# Autodesk Inventor assembly: TL20240901-10320CV-000
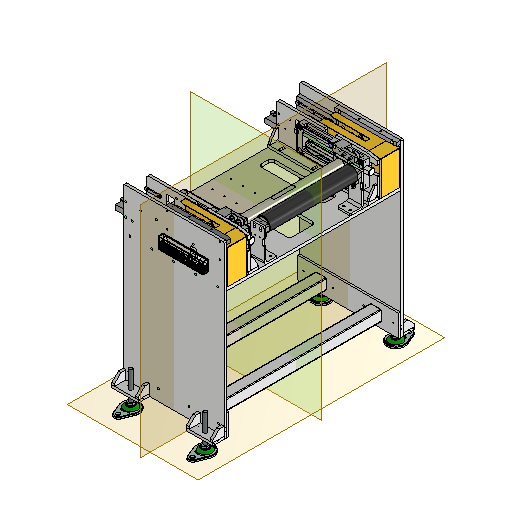
[picture p0: Inventor's stored thumbnail of the model, 512x512]
Saved by Autodesk Inventor 2022.6 (Build 266554000, 554)
## iProperties
Category: CONVEYOR ASSY
Company: 현대 트랜시스
Created: 2023-04-11
Part Number: TL20240901-10320CV-000
Checked By: 김형민
Engr Approved By: 김형민
User Status: 1 x6
Description: 5
Document SubType Name: Assembly
Mfg Approved By: 호상태
Designer: 박성규
Stock Number: 000
Project: MEa-PJT 2LINE
DocNumber: TN20221101-FA000000-000-1.iam
Folder: OLD\개발설비\1. 사내개발\19. 미쓰비시 컨버팅 솔루션 데모장비\
Detail Description: Assembly products
Title: FOLLOWER UNIT ASSY
Subject: MEa차종 시트조립2라인
Author: 박성규
Revision Number: A
## Documents named in this file (45)
- D:\V\Designs\프로젝트 자산\자동화 & 스마트팩토리\현대트랜시스(구 다이모스, 파워텍)\트랜시스(사바나)_TL20240901-MEa차종 시트조립2라인 조립컨베어 신작\2. 제작도면\1열\10300CV(CONVEYOR)\10320CV(FOLLOWER UNIT)\TL20240901-10320CV-000.iam
- D:\V\Designs\프로젝트 자산\자동화 & 스마트팩토리\현대트랜시스(구 다이모스, 파워텍)\트랜시스(사바나)_TL20240901-MEa차종 시트조립2라인 조립컨베어 신작\2. 제작도면\1열\10300CV(CONVEYOR)\10320CV(FOLLOWER UNIT)\TL20240901-10320CV-005.ipt
- D:\V\Designs\프로젝트 자산\자동화 & 스마트팩토리\현대트랜시스(구 다이모스, 파워텍)\트랜시스(사바나)_TL20240901-MEa차종 시트조립2라인 조립컨베어 신작\2. 제작도면\1열\10300CV(CONVEYOR)\10320CV(FOLLOWER UNIT)\TL20240901-10320CV-019.ipt
- D:\V\Designs\프로젝트 자산\자동화 & 스마트팩토리\현대트랜시스(구 다이모스, 파워텍)\트랜시스(사바나)_TL20240901-MEa차종 시트조립2라인 조립컨베어 신작\2. 제작도면\1열\10300CV(CONVEYOR)\10320CV(FOLLOWER UNIT)\TL20240901-10320CV-015.ipt
- D:\V\Designs\프로젝트 자산\자동화 & 스마트팩토리\현대트랜시스(구 다이모스, 파워텍)\트랜시스(사바나)_TL20240901-MEa차종 시트조립2라인 조립컨베어 신작\2. 제작도면\1열\10300CV(CONVEYOR)\10320CV(FOLLOWER UNIT)\TL20240901-10320CV-001.ipt
- D:\V\Designs\프로젝트 자산\자동화 & 스마트팩토리\현대트랜시스(구 다이모스, 파워텍)\트랜시스(사바나)_TL20240901-MEa차종 시트조립2라인 조립컨베어 신작\2. 제작도면\1열\10300CV(CONVEYOR)\10320CV(FOLLOWER UNIT)\TL20240901-10320CV-002.ipt
- D:\V\Designs\프로젝트 자산\자동화 & 스마트팩토리\현대트랜시스(구 다이모스, 파워텍)\트랜시스(사바나)_TL20240901-MEa차종 시트조립2라인 조립컨베어 신작\2. 제작도면\1열\10300CV(CONVEYOR)\10320CV(FOLLOWER UNIT)\TL20240901-10320CV-024.ipt
- D:\V\Designs\프로젝트 자산\자동화 & 스마트팩토리\현대트랜시스(구 다이모스, 파워텍)\트랜시스(사바나)_TL20240901-MEa차종 시트조립2라인 조립컨베어 신작\2. 제작도면\1열\10300CV(CONVEYOR)\10320CV(FOLLOWER UNIT)\TL20240901-10320CV-013.ipt
- D:\V\Designs\구매품(업체별)\THK\CAM FOLLOWER_CF10-1UU_THK.ipt
- D:\V\Designs\구매품(업체별)\BUYOUNG\ADJUST ANCHOR_BYARB-81-M16X130_BUYOUNG.ipt
- D:\V\Designs\프로젝트 자산\자동화 & 스마트팩토리\현대트랜시스(구 다이모스, 파워텍)\트랜시스(사바나)_TL20240901-MEa차종 시트조립2라인 조립컨베어 신작\2. 제작도면\1열\10300CV(CONVEYOR)\10320CV(FOLLOWER UNIT)\TL20240901-10320CV-014.ipt
- D:\V\Designs\프로젝트 자산\자동화 & 스마트팩토리\현대트랜시스(구 다이모스, 파워텍)\트랜시스(사바나)_TL20240901-MEa차종 시트조립2라인 조립컨베어 신작\2. 제작도면\1열\10300CV(CONVEYOR)\10320CV(FOLLOWER UNIT)\TL20240901-10320CV-014-MIR.ipt
- D:\V\Designs\프로젝트 자산\자동화 & 스마트팩토리\현대트랜시스(구 다이모스, 파워텍)\트랜시스(사바나)_TL20240901-MEa차종 시트조립2라인 조립컨베어 신작\2. 제작도면\1열\10300CV(CONVEYOR)\10320CV(FOLLOWER UNIT)\TL20240901-10320CV-022.ipt
- D:\V\Designs\프로젝트 자산\자동화 & 스마트팩토리\현대트랜시스(구 다이모스, 파워텍)\트랜시스(사바나)_TL20240901-MEa차종 시트조립2라인 조립컨베어 신작\2. 제작도면\1열\10300CV(CONVEYOR)\10320CV(FOLLOWER UNIT)\TL20240901-10320CV-023.ipt
- D:\V\Designs\구매품(업체별)\EUNHYUN\FREE ROLLER_FR570-400-12-JD-ZN-NR630A_EUNHYUN.ipt
- D:\V\Designs\프로젝트 자산\자동화 & 스마트팩토리\현대트랜시스(구 다이모스, 파워텍)\트랜시스(사바나)_TL20240901-MEa차종 시트조립2라인 조립컨베어 신작\2. 제작도면\1열\10300CV(CONVEYOR)\10320CV(FOLLOWER UNIT)\TL20240901-10320CV-008.ipt
- D:\V\Designs\프로젝트 자산\자동화 & 스마트팩토리\현대트랜시스(구 다이모스, 파워텍)\트랜시스(사바나)_TL20240901-MEa차종 시트조립2라인 조립컨베어 신작\2. 제작도면\1열\10300CV(CONVEYOR)\10320CV(FOLLOWER UNIT)\TL20240901-10320CV-007.ipt
- D:\V\Designs\구매품(업체별)\NSK\BEARING_60-32ZZ_NSK.ipt
- D:\V\Designs\프로젝트 자산\자동화 & 스마트팩토리\현대트랜시스(구 다이모스, 파워텍)\트랜시스(사바나)_TL20240901-MEa차종 시트조립2라인 조립컨베어 신작\2. 제작도면\1열\10300CV(CONVEYOR)\10320CV(FOLLOWER UNIT)\TL20240901-10320CV-010.ipt
- D:\V\Designs\프로젝트 자산\자동화 & 스마트팩토리\현대트랜시스(구 다이모스, 파워텍)\트랜시스(사바나)_TL20240901-MEa차종 시트조립2라인 조립컨베어 신작\2. 제작도면\1열\10300CV(CONVEYOR)\10320CV(FOLLOWER UNIT)\TL20240901-10320CV-006.ipt
- D:\V\Designs\프로젝트 자산\자동화 & 스마트팩토리\현대트랜시스(구 다이모스, 파워텍)\트랜시스(사바나)_TL20240901-MEa차종 시트조립2라인 조립컨베어 신작\2. 제작도면\1열\10300CV(CONVEYOR)\10320CV(FOLLOWER UNIT)\TL20240901-10320CV-009.ipt
- D:\V\Designs\프로젝트 자산\자동화 & 스마트팩토리\현대트랜시스(구 다이모스, 파워텍)\트랜시스(사바나)_TL20240901-MEa차종 시트조립2라인 조립컨베어 신작\2. 제작도면\1열\10300CV(CONVEYOR)\10320CV(FOLLOWER UNIT)\TL20240901-10320CV-002-MIR.ipt
- D:\V\Designs\프로젝트 자산\자동화 & 스마트팩토리\현대트랜시스(구 다이모스, 파워텍)\트랜시스(사바나)_TL20240901-MEa차종 시트조립2라인 조립컨베어 신작\2. 제작도면\1열\10300CV(CONVEYOR)\10320CV(FOLLOWER UNIT)\TL20240901-10320CV-005-MIR.ipt
- D:\V\Designs\프로젝트 자산\자동화 & 스마트팩토리\현대트랜시스(구 다이모스, 파워텍)\트랜시스(사바나)_TL20240901-MEa차종 시트조립2라인 조립컨베어 신작\2. 제작도면\1열\10300CV(CONVEYOR)\10320CV(FOLLOWER UNIT)\TL20240901-10320CV-011.ipt
- D:\V\Designs\구매품(업체별)\기타\TAKE UP UNIT_CTSN-9(L)_SHINWOO.iam
- D:\V\Designs\구매품(업체별)\기타\TAKE UP UNIT_CTSN-9_SHINWOO.iam
- D:\V\Designs\프로젝트 자산\자동화 & 스마트팩토리\현대트랜시스(구 다이모스, 파워텍)\트랜시스(사바나)_TL20240901-MEa차종 시트조립2라인 조립컨베어 신작\2. 제작도면\1열\10300CV(CONVEYOR)\10320CV(FOLLOWER UNIT)\TL20240901-10320CV-012.ipt
- D:\V\Content Center Files\en-US\AS 1420\AS 1420 - 1973 - M8 x 40.ipt
- D:\V\Designs\구매품(업체별)\MISUMI\ADJUST BLOCK_SNTBM8-8_MISUMI.ipt
- D:\V\Content Center Files\en-US\ANSI B 18.2.4.1 M(1)\ANSI B 18.2.4.1 M - M8 x 1.25Style 1.ipt
- D:\V\Designs\프로젝트 자산\자동화 & 스마트팩토리\현대트랜시스(구 다이모스, 파워텍)\트랜시스(사바나)_TL20240901-MEa차종 시트조립2라인 조립컨베어 신작\2. 제작도면\1열\10300CV(CONVEYOR)\10320CV(FOLLOWER UNIT)\TL20240901-10320CV-020.ipt
- D:\V\Designs\프로젝트 자산\자동화 & 스마트팩토리\현대트랜시스(구 다이모스, 파워텍)\트랜시스(사바나)_TL20240901-MEa차종 시트조립2라인 조립컨베어 신작\2. 제작도면\1열\10300CV(CONVEYOR)\10320CV(FOLLOWER UNIT)\TL20240901-10320CV-016.ipt
- D:\V\Designs\프로젝트 자산\자동화 & 스마트팩토리\현대트랜시스(구 다이모스, 파워텍)\트랜시스(사바나)_TL20240901-MEa차종 시트조립2라인 조립컨베어 신작\2. 제작도면\1열\10300CV(CONVEYOR)\10320CV(FOLLOWER UNIT)\TL20240901-10320CV-016-MIR.ipt
- D:\V\Designs\프로젝트 자산\자동화 & 스마트팩토리\현대트랜시스(구 다이모스, 파워텍)\트랜시스(사바나)_TL20240901-MEa차종 시트조립2라인 조립컨베어 신작\2. 제작도면\1열\10300CV(CONVEYOR)\10320CV(FOLLOWER UNIT)\TL20240901-10320CV-017.ipt
- D:\V\Designs\프로젝트 자산\자동화 & 스마트팩토리\현대트랜시스(구 다이모스, 파워텍)\트랜시스(사바나)_TL20240901-MEa차종 시트조립2라인 조립컨베어 신작\2. 제작도면\1열\10300CV(CONVEYOR)\10320CV(FOLLOWER UNIT)\TL20240901-10320CV-018.ipt
- D:\V\Designs\프로젝트 자산\자동화 & 스마트팩토리\현대트랜시스(구 다이모스, 파워텍)\트랜시스(사바나)_TL20240901-MEa차종 시트조립2라인 조립컨베어 신작\2. 제작도면\1열\10300CV(CONVEYOR)\10320CV(FOLLOWER UNIT)\TL20240901-10320CV-004.ipt
- D:\V\Designs\프로젝트 자산\자동화 & 스마트팩토리\현대트랜시스(구 다이모스, 파워텍)\트랜시스(사바나)_TL20240901-MEa차종 시트조립2라인 조립컨베어 신작\2. 제작도면\1열\10300CV(CONVEYOR)\10320CV(FOLLOWER UNIT)\TL20240901-10320CV-003.ipt
- D:\V\Designs\프로젝트 자산\자동화 & 스마트팩토리\현대트랜시스(구 다이모스, 파워텍)\트랜시스(사바나)_TL20240901-MEa차종 시트조립2라인 조립컨베어 신작\2. 제작도면\1열\10300CV(CONVEYOR)\10320CV(FOLLOWER UNIT)\TL20240901-10320CV-013-MIR.ipt
- D:\V\Designs\프로젝트 자산\자동화 & 스마트팩토리\현대트랜시스(구 다이모스, 파워텍)\트랜시스(사바나)_TL20240901-MEa차종 시트조립2라인 조립컨베어 신작\2. 제작도면\1열\10300CV(CONVEYOR)\10320CV(FOLLOWER UNIT)\TL20240901-10320CV-021.ipt
- D:\V\Designs\구매품(업체별)\OMRON\PROXIMITY SENSOR_E2B-M18KS08-WP-B1_OMRON.ipt
- D:\V\Designs\구매품(업체별)\BUYOUNG\END CAP_BYEC-2020P-BK_BUYOUNG.ipt
- D:\V\Designs\프로젝트 자산\자동화 & 스마트팩토리\현대트랜시스(구 다이모스, 파워텍)\트랜시스(사바나)_TL20240901-MEa차종 시트조립2라인 조립컨베어 신작\2. 제작도면\1열\10300CV(CONVEYOR)\10320CV(FOLLOWER UNIT)\TL20240901-10320CV-025.ipt
- D:\V\Designs\프로젝트 자산\자동화 & 스마트팩토리\현대트랜시스(구 다이모스, 파워텍)\트랜시스(사바나)_TL20240901-MEa차종 시트조립2라인 조립컨베어 신작\2. 제작도면\1열\10300CV(CONVEYOR)\10320CV(FOLLOWER UNIT)\TL20240901-10320CV-027.ipt
- D:\V\Designs\프로젝트 자산\자동화 & 스마트팩토리\현대트랜시스(구 다이모스, 파워텍)\트랜시스(사바나)_TL20240901-MEa차종 시트조립2라인 조립컨베어 신작\2. 제작도면\1열\10300CV(CONVEYOR)\10320CV(FOLLOWER UNIT)\TL20240901-10320CV-026.ipt
- D:\V\Designs\프로젝트 자산\자동화 & 스마트팩토리\현대트랜시스(구 다이모스, 파워텍)\트랜시스(사바나)_TL20240901-MEa차종 시트조립2라인 조립컨베어 신작\2. 제작도면\1열\10300CV(CONVEYOR)\10320CV(FOLLOWER UNIT)\TL20240901-10320CV-101.ipt
## Components (96 placed, 44 different names)
1. ADJUST ANCHOR_BYARB-81-M16X130_BUYOUNG.ipt:1 — 메이트:426, 플러쉬:20, 플러쉬:21, 각도:2, 각도:3, Flush:44
2. ADJUST ANCHOR_BYARB-81-M16X130_BUYOUNG.ipt:2 — 메이트:427, 플러쉬:21, 각도:3
3. ADJUST ANCHOR_BYARB-81-M16X130_BUYOUNG.ipt:3 — 메이트:424, 플러쉬:19, 플러쉬:20, 각도:5, Flush:22, Flush:44
4. ADJUST ANCHOR_BYARB-81-M16X130_BUYOUNG.ipt:4 — 메이트:425, 플러쉬:19, 각도:5, Mate:518
5. ADJUST BLOCK_SNTBM8-8_MISUMI.ipt:1 — Mate:586, Mate:587, Mate:588, Mate:589, Mate:590
6. ADJUST BLOCK_SNTBM8-8_MISUMI.ipt:2 — Mate:594, Mate:595, Mate:596
7. ANSI B 18.2.4.1 M - M8 x 1.25Style 1.ipt:1 — Mate:590
8. ANSI B 18.2.4.1 M - M8 x 1.25Style 1.ipt:2
9. AS 1420 - 1973 - M8 x 40.ipt:1 — Mate:589
10. AS 1420 - 1973 - M8 x 40.ipt:2 — Mate:597
11. BEARING_60-32ZZ_NSK.ipt:1
12. BEARING_60-32ZZ_NSK.ipt:2
13. BEARING_60-32ZZ_NSK.ipt:3
14. BEARING_60-32ZZ_NSK.ipt:4
15. CAM FOLLOWER_CF10-1UU_THK.ipt:1
16. CAM FOLLOWER_CF10-1UU_THK.ipt:2
17. CAM FOLLOWER_CF10-1UU_THK.ipt:3 — Mate:599, Mate:604
18. CAM FOLLOWER_CF10-1UU_THK.ipt:4 — Mate:598, Mate:603
19. END CAP_BYEC-2020P-BK_BUYOUNG.ipt:1
20. END CAP_BYEC-2020P-BK_BUYOUNG.ipt:2
21. END CAP_BYEC-2020P-BK_BUYOUNG.ipt:3
22. END CAP_BYEC-2020P-BK_BUYOUNG.ipt:4
23. FREE ROLLER_FR570-400-12-JD-ZN-NR630A_EUNHYUN.ipt:1
24. PROXIMITY SENSOR_E2B-M18KS08-WP-B1_OMRON.ipt:1
25. PROXIMITY SENSOR_E2B-M18KS08-WP-B1_OMRON.ipt:2
26. TAKE UP UNIT_CTSN-9(L)_SHINWOO.iam:1 [sub-assembly] — Mate:561, Mate:562, Mate:563, Mate:564, Mate:566, Mate:567, Mate:568, Mate:569, Mate:574, Mate:585
27. TAKE UP UNIT_CTSN-9_SHINWOO.iam:1 [sub-assembly] — Mate:565, Mate:570, Mate:571, Mate:572, Mate:573, Mate:584
28. TL20240901-10320CV-001.ipt:1 — 메이트:148, 메이트:149, 메이트:150, 메이트:194, Mate:451, Mate:452, Mate:473, Mate:508, Mate:509, Mate:510, Mate:529, Mate:530, Mate:531, Mate:532, Mate:575, Mate:580, Flush:41, Mate:582, Flush:42, Angle:6, Angle:7
29. TL20240901-10320CV-002-MIR.ipt:1 — Mate:499, Mate:500, Mate:501, Mate:502, Mate:503, Mate:504, Mate:505, Mate:506, Mate:507, Mate:508, Mate:509, Mate:510, Mate:511, Mate:512, Mate:513, Mate:514, Mate:515, Mate:516, Mate:517, Mate:519, Mate:520, Mate:581, Mate:635, Mate:636, Mate:637
30. TL20240901-10320CV-002.ipt:1 — 메이트:148, 메이트:149, 메이트:150, 메이트:206, 메이트:207, 메이트:208, 메이트:209, 메이트:210, 메이트:211, 메이트:378, 메이트:379, 메이트:380, 메이트:389, 메이트:390, 메이트:391, 각도:2, Mate:446, Mate:447, Mate:448, Mate:583, Mate:622, Mate:623, Mate:624
31. TL20240901-10320CV-003.ipt:1
32. TL20240901-10320CV-003.ipt:2
33. TL20240901-10320CV-003.ipt:3
34. TL20240901-10320CV-003.ipt:4 — 메이트:389
35. TL20240901-10320CV-003.ipt:5
36. TL20240901-10320CV-003.ipt:6 — Mate:499
37. TL20240901-10320CV-003.ipt:7
38. TL20240901-10320CV-003.ipt:8
39. TL20240901-10320CV-004.ipt:1 — 메이트:378, 메이트:379, 메이트:380, 메이트:426
40. TL20240901-10320CV-004.ipt:2 — 메이트:390, 메이트:391, 메이트:427
41. TL20240901-10320CV-004.ipt:3 — 메이트:424, Flush:22, Mate:506, Mate:507
42. TL20240901-10320CV-004.ipt:4 — 메이트:425, Mate:503, Mate:504, Mate:505
43. TL20240901-10320CV-005-MIR.ipt:1 — Mate:529, Mate:530, Mate:531, Mate:532, Mate:533, Mate:534, Mate:535, Mate:536, Mate:537, Mate:566, Mate:567, Mate:568, Mate:600, Mate:601, Mate:602
44. TL20240901-10320CV-005.ipt:1 — 메이트:194, 메이트:366, 메이트:367, Mate:451, Mate:452, Mate:528, Mate:565, Mate:570, Mate:571, Mate:605
45. TL20240901-10320CV-006.ipt:1
46. TL20240901-10320CV-006.ipt:2
47. TL20240901-10320CV-007.ipt:1 — Flush:43, Angle:7
48. TL20240901-10320CV-007.ipt:2 — Flush:43
49. TL20240901-10320CV-008.ipt:1 — Mate:572, Mate:574, Mate:575, Mate:584, Angle:6
50. TL20240901-10320CV-009.ipt:1
51. TL20240901-10320CV-009.ipt:2
52. TL20240901-10320CV-010.ipt:1 — Mate:585
53. TL20240901-10320CV-010.ipt:2 — Mate:573
54. TL20240901-10320CV-011.ipt:1
55. TL20240901-10320CV-011.ipt:2 — Mate:563, Mate:564
56. TL20240901-10320CV-011.ipt:3
57. TL20240901-10320CV-011.ipt:4
58. TL20240901-10320CV-011.ipt:5
59. TL20240901-10320CV-011.ipt:6 — Mate:569
60. TL20240901-10320CV-011.ipt:7
61. TL20240901-10320CV-011.ipt:8 — Mate:561, Mate:562
62. TL20240901-10320CV-012.ipt:1
63. TL20240901-10320CV-012.ipt:2
64. TL20240901-10320CV-013-MIR.ipt:1 — Mate:598, Mate:599, Mate:600, Mate:601, Mate:602, Mate:603, Mate:604
65. TL20240901-10320CV-013.ipt:1 — 메이트:366, 메이트:367, Mate:528
66. TL20240901-10320CV-014-MIR.ipt:1 — Mate:446, Mate:447, Mate:448
67. TL20240901-10320CV-014.ipt:1 — Mate:511, Mate:512, Mate:513
68. TL20240901-10320CV-015.ipt:1 — Mate:514, Mate:515, Mate:516
69. TL20240901-10320CV-015.ipt:2 — 메이트:209, 메이트:210, 메이트:211
70. TL20240901-10320CV-016-MIR.ipt:1 — 메이트:206, 메이트:207, 메이트:208
71. TL20240901-10320CV-016.ipt:1 — Mate:517, Mate:519, Mate:520
72. TL20240901-10320CV-017.ipt:1
73. TL20240901-10320CV-017.ipt:2
74. TL20240901-10320CV-018.ipt:1
75. TL20240901-10320CV-018.ipt:2 — Mate:536, Mate:537
76. TL20240901-10320CV-018.ipt:3
77. TL20240901-10320CV-018.ipt:4
78. TL20240901-10320CV-019.ipt:1 — Mate:605
79. TL20240901-10320CV-019.ipt:2 — Mate:533, Mate:534, Mate:535
80. TL20240901-10320CV-020.ipt:1
81. TL20240901-10320CV-020.ipt:2
82. TL20240901-10320CV-021.ipt:1 — Mate:580, Mate:581, Flush:41, Mate:607, Mate:608, Mate:609
83. TL20240901-10320CV-021.ipt:2 — Mate:582, Mate:583, Flush:42, Mate:606, Mate:610, Mate:611
84. TL20240901-10320CV-022.ipt:1 — Mate:473, Mate:586, Mate:587, Mate:588
85. TL20240901-10320CV-022.ipt:2 — Mate:594, Mate:595, Mate:596
86. TL20240901-10320CV-023.ipt:1
87. TL20240901-10320CV-023.ipt:2 — Mate:597
88. TL20240901-10320CV-024.ipt:1 — Flush:39, Flush:40, Mate:500, Mate:501, Mate:502
89. TL20240901-10320CV-025.ipt:1 — Mate:607, Mate:608, Mate:609
90. TL20240901-10320CV-025.ipt:2 — Mate:606, Mate:610, Mate:611
91. TL20240901-10320CV-026.ipt:1 — Flush:51
92. TL20240901-10320CV-026.ipt:2 — Flush:51
93. TL20240901-10320CV-027.ipt:1
94. TL20240901-10320CV-027.ipt:2
95. TL20240901-10320CV-101.ipt:1 — Mate:622, Mate:623, Mate:624
96. TL20240901-10320CV-101.ipt:2 — Mate:635, Mate:636, Mate:637
## Relationships (260: Mate 229, Flush 24, Angle 7)
- 메이트:148 [Mate]: TL20240901-10320CV-001.ipt:1 ↔ TL20240901-10320CV-002.ipt:1
- 메이트:149 [Mate]: TL20240901-10320CV-001.ipt:1 ↔ TL20240901-10320CV-002.ipt:1
- 메이트:150 [Mate]: TL20240901-10320CV-001.ipt:1 ↔ TL20240901-10320CV-002.ipt:1
- [Mate] (5 mm): TL20240901-10320CV-016.ipt:1 ↔ TL20240901-10320CV-018.ipt:4
- [Mate]: TL20240901-10320CV-016.ipt:1 ↔ TL20240901-10320CV-018.ipt:4
- [Mate]: TL20240901-10320CV-016.ipt:1 ↔ TL20240901-10320CV-018.ipt:4
- [Mate] (5 mm): TL20240901-10320CV-016.ipt:1 ↔ TL20240901-10320CV-017.ipt:1
- [Mate]: TL20240901-10320CV-016.ipt:1 ↔ TL20240901-10320CV-017.ipt:1
- [Mate]: TL20240901-10320CV-016.ipt:1 ↔ TL20240901-10320CV-017.ipt:1
- [Mate] (5 mm): TL20240901-10320CV-005.ipt:1 ↔ TL20240901-10320CV-019.ipt:1
- [Mate]: TL20240901-10320CV-005.ipt:1 ↔ TL20240901-10320CV-019.ipt:1
- [Mate] (5 mm): TL20240901-10320CV-005.ipt:1 ↔ TL20240901-10320CV-018.ipt:1
- [Mate]: TL20240901-10320CV-005.ipt:1 ↔ TL20240901-10320CV-018.ipt:1
- [Mate]: TL20240901-10320CV-005.ipt:1 ↔ TL20240901-10320CV-018.ipt:1
- [Mate] (5 mm): TL20240901-10320CV-016-MIR.ipt:1 ↔ TL20240901-10320CV-018.ipt:3
- [Mate] (5 mm): TL20240901-10320CV-016-MIR.ipt:1 ↔ TL20240901-10320CV-017.ipt:2
- [Mate]: TL20240901-10320CV-016-MIR.ipt:1 ↔ TL20240901-10320CV-018.ipt:3
- [Mate]: TL20240901-10320CV-016-MIR.ipt:1 ↔ TL20240901-10320CV-018.ipt:3
- [Mate]: TL20240901-10320CV-016-MIR.ipt:1 ↔ TL20240901-10320CV-017.ipt:2
- [Mate]: TL20240901-10320CV-016-MIR.ipt:1 ↔ TL20240901-10320CV-017.ipt:2
- 메이트:194 [Mate]: TL20240901-10320CV-001.ipt:1 ↔ TL20240901-10320CV-005.ipt:1
- [Mate]: TL20240901-10320CV-001.ipt:1 ↔ TL20240901-10320CV-022.ipt:1
- [Mate]: TL20240901-10320CV-001.ipt:1 ↔ TL20240901-10320CV-022.ipt:2
- 메이트:206 [Mate]: TL20240901-10320CV-002.ipt:1 ↔ TL20240901-10320CV-016-MIR.ipt:1
- 메이트:207 [Mate]: TL20240901-10320CV-002.ipt:1 ↔ TL20240901-10320CV-016-MIR.ipt:1
- 메이트:208 [Mate]: TL20240901-10320CV-002.ipt:1 ↔ TL20240901-10320CV-016-MIR.ipt:1
- 메이트:209 [Mate]: TL20240901-10320CV-002.ipt:1 ↔ TL20240901-10320CV-015.ipt:2
- 메이트:210 [Mate]: TL20240901-10320CV-002.ipt:1 ↔ TL20240901-10320CV-015.ipt:2
- 메이트:211 [Mate]: TL20240901-10320CV-002.ipt:1 ↔ TL20240901-10320CV-015.ipt:2
- [Mate]: CAM FOLLOWER_CF10-1UU_THK.ipt:1 ↔ TL20240901-10320CV-013.ipt:1
- [Mate]: CAM FOLLOWER_CF10-1UU_THK.ipt:1 ↔ TL20240901-10320CV-013.ipt:1
- [Mate]: CAM FOLLOWER_CF10-1UU_THK.ipt:2 ↔ TL20240901-10320CV-013.ipt:1
- [Mate]: CAM FOLLOWER_CF10-1UU_THK.ipt:2 ↔ TL20240901-10320CV-013.ipt:1
- 메이트:366 [Mate]: TL20240901-10320CV-005.ipt:1 ↔ TL20240901-10320CV-013.ipt:1
- 메이트:367 [Mate]: TL20240901-10320CV-005.ipt:1 ↔ TL20240901-10320CV-013.ipt:1
- [Mate]: TL20240901-10320CV-003.ipt:1 ↔ TL20240901-10320CV-004.ipt:1
- [Mate]: TL20240901-10320CV-003.ipt:1 ↔ TL20240901-10320CV-004.ipt:1
- [Mate]: TL20240901-10320CV-003.ipt:1 ↔ TL20240901-10320CV-004.ipt:1
- [Mate]: TL20240901-10320CV-003.ipt:2 ↔ TL20240901-10320CV-004.ipt:1
- [Mate]: TL20240901-10320CV-003.ipt:2 ↔ TL20240901-10320CV-004.ipt:1
- [Mate]: TL20240901-10320CV-003.ipt:2 ↔ TL20240901-10320CV-004.ipt:1
- 메이트:378 [Mate]: TL20240901-10320CV-002.ipt:1 ↔ TL20240901-10320CV-004.ipt:1
- 메이트:379 [Mate]: TL20240901-10320CV-002.ipt:1 ↔ TL20240901-10320CV-004.ipt:1
- 메이트:380 [Mate]: TL20240901-10320CV-002.ipt:1 ↔ TL20240901-10320CV-004.ipt:1
- [Mate]: TL20240901-10320CV-003.ipt:3 ↔ TL20240901-10320CV-004.ipt:2
- [Mate]: TL20240901-10320CV-003.ipt:3 ↔ TL20240901-10320CV-004.ipt:2
- [Mate]: TL20240901-10320CV-003.ipt:3 ↔ TL20240901-10320CV-004.ipt:2
- [Mate]: TL20240901-10320CV-003.ipt:4 ↔ TL20240901-10320CV-004.ipt:2
- [Mate]: TL20240901-10320CV-003.ipt:4 ↔ TL20240901-10320CV-004.ipt:2
- [Mate]: TL20240901-10320CV-003.ipt:4 ↔ TL20240901-10320CV-004.ipt:2
- 메이트:389 [Mate]: TL20240901-10320CV-002.ipt:1 ↔ TL20240901-10320CV-003.ipt:4
- 메이트:390 [Mate]: TL20240901-10320CV-002.ipt:1 ↔ TL20240901-10320CV-004.ipt:2
- 메이트:391 [Mate]: TL20240901-10320CV-002.ipt:1 ↔ TL20240901-10320CV-004.ipt:2
- [Mate]: TL20240901-10320CV-003.ipt:5 ↔ TL20240901-10320CV-004.ipt:3
- [Mate]: TL20240901-10320CV-003.ipt:5 ↔ TL20240901-10320CV-004.ipt:3
- [Mate]: TL20240901-10320CV-003.ipt:5 ↔ TL20240901-10320CV-004.ipt:3
- [Mate]: TL20240901-10320CV-003.ipt:6 ↔ TL20240901-10320CV-004.ipt:3
- [Mate]: TL20240901-10320CV-003.ipt:6 ↔ TL20240901-10320CV-004.ipt:3
- [Mate]: TL20240901-10320CV-003.ipt:6 ↔ TL20240901-10320CV-004.ipt:3
- [Mate]: TL20240901-10320CV-003.ipt:7 ↔ TL20240901-10320CV-004.ipt:4
- [Mate]: TL20240901-10320CV-003.ipt:7 ↔ TL20240901-10320CV-004.ipt:4
- [Mate]: TL20240901-10320CV-003.ipt:7 ↔ TL20240901-10320CV-004.ipt:4
- [Mate]: TL20240901-10320CV-003.ipt:8 ↔ TL20240901-10320CV-004.ipt:4
- [Mate]: TL20240901-10320CV-003.ipt:8 ↔ TL20240901-10320CV-004.ipt:4
- [Mate]: TL20240901-10320CV-003.ipt:8 ↔ TL20240901-10320CV-004.ipt:4
- 메이트:424 [Mate]: ADJUST ANCHOR_BYARB-81-M16X130_BUYOUNG.ipt:3 ↔ TL20240901-10320CV-004.ipt:3
- 메이트:425 [Mate]: ADJUST ANCHOR_BYARB-81-M16X130_BUYOUNG.ipt:4 ↔ TL20240901-10320CV-004.ipt:4
- 플러쉬:19 [Flush]: ADJUST ANCHOR_BYARB-81-M16X130_BUYOUNG.ipt:3 ↔ ADJUST ANCHOR_BYARB-81-M16X130_BUYOUNG.ipt:4
- 메이트:426 [Mate]: ADJUST ANCHOR_BYARB-81-M16X130_BUYOUNG.ipt:1 ↔ TL20240901-10320CV-004.ipt:1
- 플러쉬:20 [Flush]: ADJUST ANCHOR_BYARB-81-M16X130_BUYOUNG.ipt:1 ↔ ADJUST ANCHOR_BYARB-81-M16X130_BUYOUNG.ipt:3
- 메이트:427 [Mate]: ADJUST ANCHOR_BYARB-81-M16X130_BUYOUNG.ipt:2 ↔ TL20240901-10320CV-004.ipt:2
- 플러쉬:21 [Flush]: ADJUST ANCHOR_BYARB-81-M16X130_BUYOUNG.ipt:1 ↔ ADJUST ANCHOR_BYARB-81-M16X130_BUYOUNG.ipt:2
- 각도:2 [Angle] (180 deg): ADJUST ANCHOR_BYARB-81-M16X130_BUYOUNG.ipt:1 ↔ TL20240901-10320CV-002.ipt:1
- 각도:3 [Angle] (0 deg): ADJUST ANCHOR_BYARB-81-M16X130_BUYOUNG.ipt:1 ↔ ADJUST ANCHOR_BYARB-81-M16X130_BUYOUNG.ipt:2
- 각도:5 [Angle] (0 deg): ADJUST ANCHOR_BYARB-81-M16X130_BUYOUNG.ipt:3 ↔ ADJUST ANCHOR_BYARB-81-M16X130_BUYOUNG.ipt:4
- Flush:22 (66 mm): ADJUST ANCHOR_BYARB-81-M16X130_BUYOUNG.ipt:3 ↔ TL20240901-10320CV-004.ipt:3
- Mate:446: TL20240901-10320CV-002.ipt:1 ↔ TL20240901-10320CV-014-MIR.ipt:1
- Mate:447: TL20240901-10320CV-002.ipt:1 ↔ TL20240901-10320CV-014-MIR.ipt:1
- Mate:448: TL20240901-10320CV-002.ipt:1 ↔ TL20240901-10320CV-014-MIR.ipt:1
- Mate:451: TL20240901-10320CV-001.ipt:1 ↔ TL20240901-10320CV-005.ipt:1
- Mate:452: TL20240901-10320CV-001.ipt:1 ↔ TL20240901-10320CV-005.ipt:1
- [Mate]: TL20240901-10320CV-022.ipt:1 ↔ TL20240901-10320CV-023.ipt:1
- [Flush]: TL20240901-10320CV-022.ipt:1 ↔ TL20240901-10320CV-023.ipt:1
- [Flush]: TL20240901-10320CV-022.ipt:1 ↔ TL20240901-10320CV-023.ipt:1
- [Mate]: FREE ROLLER_FR570-400-12-JD-ZN-NR630A_EUNHYUN.ipt:1 ↔ TL20240901-10320CV-023.ipt:1
- [Mate]: FREE ROLLER_FR570-400-12-JD-ZN-NR630A_EUNHYUN.ipt:1 ↔ TL20240901-10320CV-023.ipt:1
- [Mate]: TL20240901-10320CV-022.ipt:2 ↔ TL20240901-10320CV-023.ipt:2
- [Flush]: TL20240901-10320CV-022.ipt:2 ↔ TL20240901-10320CV-023.ipt:2
- [Flush]: TL20240901-10320CV-022.ipt:2 ↔ TL20240901-10320CV-023.ipt:2
- [Mate]: FREE ROLLER_FR570-400-12-JD-ZN-NR630A_EUNHYUN.ipt:1 ↔ TL20240901-10320CV-023.ipt:2
- [Mate]: FREE ROLLER_FR570-400-12-JD-ZN-NR630A_EUNHYUN.ipt:1 ↔ TL20240901-10320CV-023.ipt:2
- [Flush]: TL20240901-10320CV-022.ipt:1 ↔ TL20240901-10320CV-022.ipt:2
- [Mate]: ANSI B 18.2.4.1 M - M8 x 1.25Style 1.ipt:1 ↔ AS 1420 - 1973 - M8 x 40.ipt:1
- [Mate]: AS 1420 - 1973 - M8 x 40.ipt:1 ↔ TL20240901-10320CV-023.ipt:1
- Mate:473: TL20240901-10320CV-001.ipt:1 ↔ TL20240901-10320CV-022.ipt:1
- [Mate]: BEARING_60-32ZZ_NSK.ipt:1 ↔ TL20240901-10320CV-007.ipt:1
- [Mate]: BEARING_60-32ZZ_NSK.ipt:1 ↔ TL20240901-10320CV-007.ipt:1
- [Mate]: BEARING_60-32ZZ_NSK.ipt:2 ↔ TL20240901-10320CV-007.ipt:1
- [Mate]: BEARING_60-32ZZ_NSK.ipt:2 ↔ TL20240901-10320CV-007.ipt:1
- [Mate]: BEARING_60-32ZZ_NSK.ipt:3 ↔ TL20240901-10320CV-007.ipt:2
- [Mate]: BEARING_60-32ZZ_NSK.ipt:3 ↔ TL20240901-10320CV-007.ipt:2
- [Mate]: BEARING_60-32ZZ_NSK.ipt:4 ↔ TL20240901-10320CV-007.ipt:2
- [Mate]: BEARING_60-32ZZ_NSK.ipt:4 ↔ TL20240901-10320CV-007.ipt:2
- [Mate]: TL20240901-10320CV-008.ipt:1 ↔ TL20240901-10320CV-010.ipt:1
- [Mate]: TL20240901-10320CV-008.ipt:1 ↔ TL20240901-10320CV-010.ipt:2
- [Mate]: BEARING_60-32ZZ_NSK.ipt:3 ↔ TL20240901-10320CV-010.ipt:2
- [Mate]: TL20240901-10320CV-007.ipt:2 ↔ TL20240901-10320CV-008.ipt:1
- [Mate]: BEARING_60-32ZZ_NSK.ipt:1 ↔ TL20240901-10320CV-010.ipt:1
- [Mate]: TL20240901-10320CV-007.ipt:1 ↔ TL20240901-10320CV-008.ipt:1
- [Mate]: BEARING_60-32ZZ_NSK.ipt:2 ↔ TL20240901-10320CV-006.ipt:1
- [Mate]: TL20240901-10320CV-006.ipt:1 ↔ TL20240901-10320CV-008.ipt:1
- [Mate]: BEARING_60-32ZZ_NSK.ipt:4 ↔ TL20240901-10320CV-006.ipt:2
- [Mate]: TL20240901-10320CV-006.ipt:2 ↔ TL20240901-10320CV-007.ipt:2
- [Mate]: TL20240901-10320CV-008.ipt:1 ↔ TL20240901-10320CV-009.ipt:1
- [Flush]: TL20240901-10320CV-007.ipt:2 ↔ TL20240901-10320CV-009.ipt:1
- [Mate]: TL20240901-10320CV-008.ipt:1 ↔ TL20240901-10320CV-009.ipt:2
- [Flush]: TL20240901-10320CV-007.ipt:1 ↔ TL20240901-10320CV-009.ipt:2
- Flush:39: TL20240901-10320CV-024.ipt:1
- Flush:40: TL20240901-10320CV-024.ipt:1
- Mate:499: TL20240901-10320CV-002-MIR.ipt:1 ↔ TL20240901-10320CV-003.ipt:6
- Mate:500: TL20240901-10320CV-002-MIR.ipt:1 ↔ TL20240901-10320CV-024.ipt:1
- Mate:501: TL20240901-10320CV-002-MIR.ipt:1 ↔ TL20240901-10320CV-024.ipt:1
- Mate:502: TL20240901-10320CV-002-MIR.ipt:1 ↔ TL20240901-10320CV-024.ipt:1
- Mate:503: TL20240901-10320CV-002-MIR.ipt:1 ↔ TL20240901-10320CV-004.ipt:4
- Mate:504: TL20240901-10320CV-002-MIR.ipt:1 ↔ TL20240901-10320CV-004.ipt:4
- Mate:505: TL20240901-10320CV-002-MIR.ipt:1 ↔ TL20240901-10320CV-004.ipt:4
- Mate:506: TL20240901-10320CV-002-MIR.ipt:1 ↔ TL20240901-10320CV-004.ipt:3
- Mate:507: TL20240901-10320CV-002-MIR.ipt:1 ↔ TL20240901-10320CV-004.ipt:3
- Mate:508: TL20240901-10320CV-001.ipt:1 ↔ TL20240901-10320CV-002-MIR.ipt:1
- Mate:509: TL20240901-10320CV-001.ipt:1 ↔ TL20240901-10320CV-002-MIR.ipt:1
- Mate:510: TL20240901-10320CV-001.ipt:1 ↔ TL20240901-10320CV-002-MIR.ipt:1
- Mate:511: TL20240901-10320CV-002-MIR.ipt:1 ↔ TL20240901-10320CV-014.ipt:1
- Mate:512: TL20240901-10320CV-002-MIR.ipt:1 ↔ TL20240901-10320CV-014.ipt:1
- Mate:513: TL20240901-10320CV-002-MIR.ipt:1 ↔ TL20240901-10320CV-014.ipt:1
- Mate:514: TL20240901-10320CV-002-MIR.ipt:1 ↔ TL20240901-10320CV-015.ipt:1
- Mate:515: TL20240901-10320CV-002-MIR.ipt:1 ↔ TL20240901-10320CV-015.ipt:1
- Mate:516: TL20240901-10320CV-002-MIR.ipt:1 ↔ TL20240901-10320CV-015.ipt:1
- Mate:517: TL20240901-10320CV-002-MIR.ipt:1 ↔ TL20240901-10320CV-016.ipt:1
- Mate:518: ADJUST ANCHOR_BYARB-81-M16X130_BUYOUNG.ipt:4
- Mate:519: TL20240901-10320CV-002-MIR.ipt:1 ↔ TL20240901-10320CV-016.ipt:1
- Mate:520: TL20240901-10320CV-002-MIR.ipt:1 ↔ TL20240901-10320CV-016.ipt:1
- Mate:528: TL20240901-10320CV-005.ipt:1 ↔ TL20240901-10320CV-013.ipt:1
- Mate:529: TL20240901-10320CV-001.ipt:1 ↔ TL20240901-10320CV-005-MIR.ipt:1
- Mate:530: TL20240901-10320CV-001.ipt:1 ↔ TL20240901-10320CV-005-MIR.ipt:1
- Mate:531: TL20240901-10320CV-001.ipt:1 ↔ TL20240901-10320CV-005-MIR.ipt:1
- Mate:532: TL20240901-10320CV-001.ipt:1 ↔ TL20240901-10320CV-005-MIR.ipt:1
- Mate:533 (5 mm): TL20240901-10320CV-005-MIR.ipt:1 ↔ TL20240901-10320CV-019.ipt:2
- Mate:534: TL20240901-10320CV-005-MIR.ipt:1 ↔ TL20240901-10320CV-019.ipt:2
- Mate:535: TL20240901-10320CV-005-MIR.ipt:1 ↔ TL20240901-10320CV-019.ipt:2
- Mate:536: TL20240901-10320CV-005-MIR.ipt:1 ↔ TL20240901-10320CV-018.ipt:2
- Mate:537 (5 mm): TL20240901-10320CV-005-MIR.ipt:1 ↔ TL20240901-10320CV-018.ipt:2
- [Mate]: TAKE UP UNIT_CTSN-9(L)_SHINWOO.iam:1 ↔ TL20240901-10320CV-011.ipt:6
- [Mate]: TAKE UP UNIT_CTSN-9(L)_SHINWOO.iam:1 ↔ TL20240901-10320CV-011.ipt:7
- [Mate]: TAKE UP UNIT_CTSN-9(L)_SHINWOO.iam:1 ↔ TL20240901-10320CV-011.ipt:7
- [Mate]: TAKE UP UNIT_CTSN-9_SHINWOO.iam:1 ↔ TL20240901-10320CV-011.ipt:4
- [Mate]: TAKE UP UNIT_CTSN-9_SHINWOO.iam:1 ↔ TL20240901-10320CV-011.ipt:4
- [Mate]: TAKE UP UNIT_CTSN-9_SHINWOO.iam:1 ↔ TL20240901-10320CV-011.ipt:3
- [Mate]: TL20240901-10320CV-011.ipt:3 ↔ TL20240901-10320CV-012.ipt:2
- [Mate]: TL20240901-10320CV-011.ipt:3 ↔ TL20240901-10320CV-012.ipt:2
- [Mate]: TAKE UP UNIT_CTSN-9_SHINWOO.iam:1 ↔ TL20240901-10320CV-011.ipt:3
- [Mate]: TAKE UP UNIT_CTSN-9_SHINWOO.iam:1 ↔ TL20240901-10320CV-011.ipt:1
- [Mate]: TAKE UP UNIT_CTSN-9_SHINWOO.iam:1 ↔ TL20240901-10320CV-011.ipt:1
- [Mate]: TAKE UP UNIT_CTSN-9_SHINWOO.iam:1 ↔ TL20240901-10320CV-011.ipt:5
- [Mate]: TAKE UP UNIT_CTSN-9_SHINWOO.iam:1 ↔ TL20240901-10320CV-011.ipt:5
- [Mate]: TL20240901-10320CV-011.ipt:4 ↔ TL20240901-10320CV-012.ipt:2
- [Mate]: TL20240901-10320CV-011.ipt:7 ↔ TL20240901-10320CV-012.ipt:1
- [Mate]: TL20240901-10320CV-011.ipt:7 ↔ TL20240901-10320CV-012.ipt:1
- [Mate]: TL20240901-10320CV-011.ipt:6 ↔ TL20240901-10320CV-012.ipt:1
- Mate:561: TAKE UP UNIT_CTSN-9(L)_SHINWOO.iam:1 ↔ TL20240901-10320CV-011.ipt:8
- Mate:562: TAKE UP UNIT_CTSN-9(L)_SHINWOO.iam:1 ↔ TL20240901-10320CV-011.ipt:8
- Mate:563: TAKE UP UNIT_CTSN-9(L)_SHINWOO.iam:1 ↔ TL20240901-10320CV-011.ipt:2
- Mate:564: TAKE UP UNIT_CTSN-9(L)_SHINWOO.iam:1 ↔ TL20240901-10320CV-011.ipt:2
- Mate:565: TAKE UP UNIT_CTSN-9_SHINWOO.iam:1 ↔ TL20240901-10320CV-005.ipt:1
- Mate:566: TAKE UP UNIT_CTSN-9(L)_SHINWOO.iam:1 ↔ TL20240901-10320CV-005-MIR.ipt:1
- Mate:567: TAKE UP UNIT_CTSN-9(L)_SHINWOO.iam:1 ↔ TL20240901-10320CV-005-MIR.ipt:1
- Mate:568: TAKE UP UNIT_CTSN-9(L)_SHINWOO.iam:1 ↔ TL20240901-10320CV-005-MIR.ipt:1
- Mate:569: TAKE UP UNIT_CTSN-9(L)_SHINWOO.iam:1 ↔ TL20240901-10320CV-011.ipt:6
- Mate:570: TAKE UP UNIT_CTSN-9_SHINWOO.iam:1 ↔ TL20240901-10320CV-005.ipt:1
- Mate:571: TAKE UP UNIT_CTSN-9_SHINWOO.iam:1 ↔ TL20240901-10320CV-005.ipt:1
- Mate:572: TAKE UP UNIT_CTSN-9_SHINWOO.iam:1 ↔ TL20240901-10320CV-008.ipt:1
- Mate:573: TAKE UP UNIT_CTSN-9_SHINWOO.iam:1 ↔ TL20240901-10320CV-010.ipt:2
- Mate:574: TAKE UP UNIT_CTSN-9(L)_SHINWOO.iam:1 ↔ TL20240901-10320CV-008.ipt:1
- Mate:575 (-140 mm): TL20240901-10320CV-001.ipt:1 ↔ TL20240901-10320CV-008.ipt:1
- [Mate]: TL20240901-10320CV-020.ipt:1 ↔ TL20240901-10320CV-021.ipt:1
- [Mate]: TL20240901-10320CV-020.ipt:1 ↔ TL20240901-10320CV-021.ipt:1
- [Mate]: TL20240901-10320CV-020.ipt:2 ↔ TL20240901-10320CV-021.ipt:2
- [Mate]: TL20240901-10320CV-020.ipt:2 ↔ TL20240901-10320CV-021.ipt:2
- Mate:580 (27 mm): TL20240901-10320CV-001.ipt:1 ↔ TL20240901-10320CV-021.ipt:1
- Mate:581 (25 mm): TL20240901-10320CV-002-MIR.ipt:1 ↔ TL20240901-10320CV-021.ipt:1
- Flush:41 (75 mm): TL20240901-10320CV-001.ipt:1 ↔ TL20240901-10320CV-021.ipt:1
- Mate:582 (27 mm): TL20240901-10320CV-001.ipt:1 ↔ TL20240901-10320CV-021.ipt:2
- Mate:583 (25 mm): TL20240901-10320CV-002.ipt:1 ↔ TL20240901-10320CV-021.ipt:2
- Flush:42 (75 mm): TL20240901-10320CV-001.ipt:1 ↔ TL20240901-10320CV-021.ipt:2
- Mate:584: TAKE UP UNIT_CTSN-9_SHINWOO.iam:1 ↔ TL20240901-10320CV-008.ipt:1
- Mate:585: TAKE UP UNIT_CTSN-9(L)_SHINWOO.iam:1 ↔ TL20240901-10320CV-010.ipt:1
- Angle:6 (0 deg): TL20240901-10320CV-001.ipt:1 ↔ TL20240901-10320CV-008.ipt:1
- Flush:43: TL20240901-10320CV-007.ipt:1 ↔ TL20240901-10320CV-007.ipt:2
- Angle:7 (0 deg): TL20240901-10320CV-001.ipt:1 ↔ TL20240901-10320CV-007.ipt:1
- Mate:586: ADJUST BLOCK_SNTBM8-8_MISUMI.ipt:1 ↔ TL20240901-10320CV-022.ipt:1
- Mate:587: ADJUST BLOCK_SNTBM8-8_MISUMI.ipt:1 ↔ TL20240901-10320CV-022.ipt:1
- Mate:588: ADJUST BLOCK_SNTBM8-8_MISUMI.ipt:1 ↔ TL20240901-10320CV-022.ipt:1
- Mate:589: ADJUST BLOCK_SNTBM8-8_MISUMI.ipt:1 ↔ AS 1420 - 1973 - M8 x 40.ipt:1
- Mate:590: ADJUST BLOCK_SNTBM8-8_MISUMI.ipt:1 ↔ ANSI B 18.2.4.1 M - M8 x 1.25Style 1.ipt:1
- [Mate]: ANSI B 18.2.4.1 M - M8 x 1.25Style 1.ipt:2 ↔ AS 1420 - 1973 - M8 x 40.ipt:2
- [Mate]: ADJUST BLOCK_SNTBM8-8_MISUMI.ipt:2 ↔ AS 1420 - 1973 - M8 x 40.ipt:2
- [Mate]: ADJUST BLOCK_SNTBM8-8_MISUMI.ipt:2 ↔ ANSI B 18.2.4.1 M - M8 x 1.25Style 1.ipt:2
- Mate:594: ADJUST BLOCK_SNTBM8-8_MISUMI.ipt:2 ↔ TL20240901-10320CV-022.ipt:2
- Mate:595: ADJUST BLOCK_SNTBM8-8_MISUMI.ipt:2 ↔ TL20240901-10320CV-022.ipt:2
- Mate:596: ADJUST BLOCK_SNTBM8-8_MISUMI.ipt:2 ↔ TL20240901-10320CV-022.ipt:2
- Mate:597: AS 1420 - 1973 - M8 x 40.ipt:2 ↔ TL20240901-10320CV-023.ipt:2
- Mate:598: CAM FOLLOWER_CF10-1UU_THK.ipt:4 ↔ TL20240901-10320CV-013-MIR.ipt:1
- Mate:599: CAM FOLLOWER_CF10-1UU_THK.ipt:3 ↔ TL20240901-10320CV-013-MIR.ipt:1
- Mate:600: TL20240901-10320CV-005-MIR.ipt:1 ↔ TL20240901-10320CV-013-MIR.ipt:1
- Mate:601: TL20240901-10320CV-005-MIR.ipt:1 ↔ TL20240901-10320CV-013-MIR.ipt:1
- Mate:602: TL20240901-10320CV-005-MIR.ipt:1 ↔ TL20240901-10320CV-013-MIR.ipt:1
- Mate:603: CAM FOLLOWER_CF10-1UU_THK.ipt:4 ↔ TL20240901-10320CV-013-MIR.ipt:1
- Mate:604: CAM FOLLOWER_CF10-1UU_THK.ipt:3 ↔ TL20240901-10320CV-013-MIR.ipt:1
- Mate:605: TL20240901-10320CV-005.ipt:1 ↔ TL20240901-10320CV-019.ipt:1
- Flush:44: ADJUST ANCHOR_BYARB-81-M16X130_BUYOUNG.ipt:1 ↔ ADJUST ANCHOR_BYARB-81-M16X130_BUYOUNG.ipt:3
- Mate:606 (5 mm): TL20240901-10320CV-021.ipt:2 ↔ TL20240901-10320CV-025.ipt:2
- Mate:607 (5 mm): TL20240901-10320CV-021.ipt:1 ↔ TL20240901-10320CV-025.ipt:1
- Mate:608: TL20240901-10320CV-021.ipt:1 ↔ TL20240901-10320CV-025.ipt:1
- Mate:609: TL20240901-10320CV-021.ipt:1 ↔ TL20240901-10320CV-025.ipt:1
- Mate:610: TL20240901-10320CV-021.ipt:2 ↔ TL20240901-10320CV-025.ipt:2
- Mate:611: TL20240901-10320CV-021.ipt:2 ↔ TL20240901-10320CV-025.ipt:2
- [Flush]: TL20240901-10320CV-026.ipt:1 ↔ TL20240901-10320CV-101.ipt:1
- [Mate]: TL20240901-10320CV-026.ipt:1 ↔ TL20240901-10320CV-101.ipt:1
- [Mate]: PROXIMITY SENSOR_E2B-M18KS08-WP-B1_OMRON.ipt:1 ↔ TL20240901-10320CV-026.ipt:1
- [Flush]: PROXIMITY SENSOR_E2B-M18KS08-WP-B1_OMRON.ipt:1 ↔ TL20240901-10320CV-026.ipt:1
- [Flush]: TL20240901-10320CV-026.ipt:1 ↔ TL20240901-10320CV-101.ipt:1
- [Mate]: TL20240901-10320CV-027.ipt:1 ↔ TL20240901-10320CV-101.ipt:1
- [Mate]: TL20240901-10320CV-027.ipt:1 ↔ TL20240901-10320CV-101.ipt:1
- [Mate]: TL20240901-10320CV-027.ipt:1 ↔ TL20240901-10320CV-101.ipt:1
- [Mate]: END CAP_BYEC-2020P-BK_BUYOUNG.ipt:1 ↔ TL20240901-10320CV-101.ipt:1
- [Mate]: END CAP_BYEC-2020P-BK_BUYOUNG.ipt:1 ↔ TL20240901-10320CV-101.ipt:1
- [Angle] (90 deg): END CAP_BYEC-2020P-BK_BUYOUNG.ipt:1 ↔ TL20240901-10320CV-101.ipt:1
- [Mate]: END CAP_BYEC-2020P-BK_BUYOUNG.ipt:2 ↔ TL20240901-10320CV-101.ipt:1
- [Mate]: END CAP_BYEC-2020P-BK_BUYOUNG.ipt:2 ↔ TL20240901-10320CV-101.ipt:1
- [Mate]: END CAP_BYEC-2020P-BK_BUYOUNG.ipt:1 ↔ END CAP_BYEC-2020P-BK_BUYOUNG.ipt:2
- Mate:622: TL20240901-10320CV-002.ipt:1 ↔ TL20240901-10320CV-101.ipt:1
- Mate:623: TL20240901-10320CV-002.ipt:1 ↔ TL20240901-10320CV-101.ipt:1
- Mate:624: TL20240901-10320CV-002.ipt:1 ↔ TL20240901-10320CV-101.ipt:1
- [Flush]: TL20240901-10320CV-026.ipt:2 ↔ TL20240901-10320CV-101.ipt:2
- [Mate]: TL20240901-10320CV-026.ipt:2 ↔ TL20240901-10320CV-101.ipt:2
- [Mate]: PROXIMITY SENSOR_E2B-M18KS08-WP-B1_OMRON.ipt:2 ↔ TL20240901-10320CV-026.ipt:2
- [Flush]: PROXIMITY SENSOR_E2B-M18KS08-WP-B1_OMRON.ipt:2 ↔ TL20240901-10320CV-026.ipt:2
- [Flush]: TL20240901-10320CV-026.ipt:2 ↔ TL20240901-10320CV-101.ipt:2
- [Mate]: TL20240901-10320CV-027.ipt:2 ↔ TL20240901-10320CV-101.ipt:2
- [Mate]: TL20240901-10320CV-027.ipt:2 ↔ TL20240901-10320CV-101.ipt:2
- [Mate]: TL20240901-10320CV-027.ipt:2 ↔ TL20240901-10320CV-101.ipt:2
- [Mate]: END CAP_BYEC-2020P-BK_BUYOUNG.ipt:3 ↔ TL20240901-10320CV-101.ipt:2
- [Mate]: END CAP_BYEC-2020P-BK_BUYOUNG.ipt:3 ↔ TL20240901-10320CV-101.ipt:2
- [Angle] (90 deg): END CAP_BYEC-2020P-BK_BUYOUNG.ipt:3 ↔ TL20240901-10320CV-101.ipt:2
- [Mate]: END CAP_BYEC-2020P-BK_BUYOUNG.ipt:4 ↔ TL20240901-10320CV-101.ipt:2
- [Mate]: END CAP_BYEC-2020P-BK_BUYOUNG.ipt:4 ↔ TL20240901-10320CV-101.ipt:2
- [Mate]: END CAP_BYEC-2020P-BK_BUYOUNG.ipt:3 ↔ END CAP_BYEC-2020P-BK_BUYOUNG.ipt:4
- Mate:635: TL20240901-10320CV-002-MIR.ipt:1 ↔ TL20240901-10320CV-101.ipt:2
- Mate:636: TL20240901-10320CV-002-MIR.ipt:1 ↔ TL20240901-10320CV-101.ipt:2
- Mate:637: TL20240901-10320CV-002-MIR.ipt:1 ↔ TL20240901-10320CV-101.ipt:2
- Flush:51: TL20240901-10320CV-026.ipt:1 ↔ TL20240901-10320CV-026.ipt:2
## Named parameters: d1490_d1604_d1327 = 5 mm, d1491_d1605_d1328 = 5 mm, d1492_d1606_d1329 = 0 mm, d1493_d1607_d1330 = 0 mm, d1494_d1608_d1331 = 0 mm, d1495_d1609_d1332 = 0 mm, d1500_d1559 = 5 mm, d1501_d1560 = 0 mm, d1502_d1561 = 0 mm, d1525_d1556 = 5 mm, d1526_d1557 = 0 mm, d1527_d1336_d1321 = 5 mm, d1528_d1337_d1322 = 0 mm, d1529_d1338_d1323 = 0 mm, d1530_d1339_d1324 = 5 mm, d1531_d1340_d1325 = 0 mm, d1532_d1341_d1326 = 0 mm, d1672_d1692_d1821_d1807 = 0 mm, d1673_d1693_d1822_d1808 = 0 mm, d1674_d1694_d1823_d1809 = 0 mm, d1675_d1695_d1824_d1818 = 0 mm, d1676_d1696_d1825_d1819 = 0 mm, d1677_d1697_d1826_d1820 = 0 mm, d1786_d1672_d1692_d1821_d1807 = 0 mm, d1787_d1673_d1693_d1822_d1808 = 0 mm, d1788_d1674_d1694_d1823_d1809 = 0 mm, d1789_d1675_d1695_d1824_d1818 = 0 mm, d1794_d1676_d1696_d1825_d1819 = 0 mm, d1795_d1677_d1697_d1826_d1820 = 0 mm, d1805_d1672_d1692_d1821_d1807 = 0 mm, d1806_d1673_d1693_d1822_d1808 = 0 mm, d1807_d1674_d1694_d1823_d1809 = 0 mm, d1808_d1675_d1695_d1824_d1818 = 0 mm, d1809_d1676_d1696_d1825_d1819 = 0 mm, d1810_d1677_d1697_d1826_d1820 = 0 mm, d1817_d1805_d1672_d1692_d1821_d1807 = 0 mm, d1818_d1806_d1673_d1693_d1822_d1808 = 0 mm, d1819_d1807_d1674_d1694_d1823_d1809 = 0 mm, d1820_d1808_d1675_d1695_d1824_d1818 = 0 mm, d1821_d1809_d1676_d1696_d1825_d1819 = 0 mm, d1822_d1810_d1677_d1697_d1826_d1820 = 0 mm, d1352_d1341 = 0 mm, d1353_d1342 = 0 mm, d1354_d1343 = 0 mm, d1531_d1527 = 0 mm, d1532_d1528 = 0 mm, d1533_d1529 = 0 mm, d1534_d1530 = 0 mm, d1909_d1538 = 0 mm, d1913_d1542 = 0 mm, d1922_d1348 = 0 mm, d1924_d1350 = 0 mm, d1925_d1351 = 0 mm, d1927_d1543 = 0 mm, d1928_d1544 = 0 mm, d1929_d1545 = 0 mm, d1930_d1546 = 0 mm, d1931_d1547 = 0 mm, d1932_d1548 = 0 mm, d1933_d1549 = 0 mm, d2367_d2674 = 0 mm, d2368_d2359 = 0 mm, d2021_d2367_d2674 = 0 mm, d2022_d2368_d2359 = 0 mm, R1 = 27 mm, R2 = 25 mm, R3 = 75 mm, d2039_d1367 = 0 mm, d2040_d2037 = 0 mm, d2041_d2038 = 0 mm, d2086_d2603 = 0 mm, d2087_d2604 = 0 mm, d2088_d2605 = 0 mm, d2089_d2606 = 0 mm, d2090_d2607 = 0 mm, d2091_d2608 = 146 mm, d2092_d2609 = 0 mm, d2093_d2610 = 0 mm, d2094_d2636 = 0 mm, d2095_d2638 = 0 mm, d2096_d2641 = 0 mm, d2097_d2642 = 0 mm, d2098_d2643 = 90 deg, d2099_d2644 = 0 mm, d2100_d2645 = 0 mm, d2101_d2646 = 0 mm
